# Autodesk Inventor assembly: StepperSystem
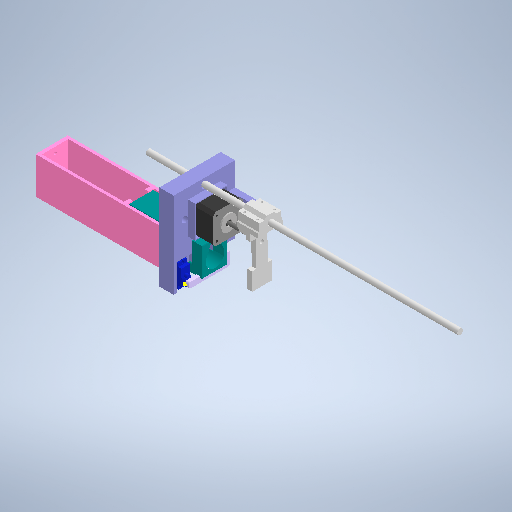
[picture p0: Inventor's stored thumbnail of the model, 512x512]
Saved by Autodesk Inventor 2025.1 (Build 291241000, 241)
## iProperties
Created: 2025-01-26
Part Number: StepperSystem
Document SubType Name: Assembly
Designer: 13156
Author: 13156
## Documents named in this file (10)
- C:\Users\13156\OneDrive - Binghamton University\Documents\GitHub\Perovskite-Automated-Synthesis-System\CAD\Pipette\StepperSystem.iam
- C:\Users\13156\OneDrive - Binghamton University\Documents\GitHub\Perovskite-Automated-Synthesis-System\CAD\Pipette\HolderWStepper.ipt
- C:\Users\13156\OneDrive - Binghamton University\Documents\GitHub\Perovskite-Automated-Synthesis-System\CAD\Non 3D Printed Parts\Motors and Servos\NEMA17 Stepper Motor.ipt
- C:\Users\13156\OneDrive - Binghamton University\Documents\GitHub\Perovskite-Automated-Synthesis-System\CAD\Non 3D Printed Parts\Linear Rails\8mm Linear Rod.ipt
- C:\Users\13156\OneDrive - Binghamton University\Documents\GitHub\Perovskite-Automated-Synthesis-System\CAD\Non 3D Printed Parts\Linear Rails\Linear Bearing 8mm Square.ipt
- C:\Users\13156\OneDrive - Binghamton University\Documents\GitHub\Perovskite-Automated-Synthesis-System\CAD\Pipette\Actuator.ipt
- C:\Users\13156\OneDrive - Binghamton University\Documents\GitHub\Perovskite-Automated-Synthesis-System\CAD\Pipette\PipetteSleeveFullLength.ipt
- C:\Users\13156\OneDrive - Binghamton University\Documents\GitHub\Perovskite-Automated-Synthesis-System\CAD\Pipette\PipetteStand.ipt
- C:\Users\13156\OneDrive - Binghamton University\Documents\GitHub\Perovskite-Automated-Synthesis-System\CAD\Non 3D Printed Parts\Motors and Servos\SG90 Servo.ipt
- C:\Users\13156\OneDrive - Binghamton University\Documents\GitHub\Perovskite-Automated-Synthesis-System\CAD\Pipette\GrabberArm.ipt
## Components (9 placed, 9 different names)
1. HolderWStepper:1 — Mate:1, Angle:1, Mate:4
2. NEMA17 Stepper Motor:1 — Mate:1
3. 8mm Linear Rod:1 — Angle:1, Mate:2
4. Linear Bearing 8mm Square:1 — Mate:2
5. Actuator:1
6. PipetteSleeveFullLength:1 — Mate:3
7. PipetteStand:1 — Mate:3
8. SG90 Servo:1 — Mate:4, Mate:5, Mate:6
9. GrabberArm:1 — Mate:5, Mate:6
## Relationships (7: Mate 6, Angle 1)
- Mate:1: HolderWStepper:1 ↔ NEMA17 Stepper Motor:1
- Angle:1 (0 deg): HolderWStepper:1 ↔ 8mm Linear Rod:1
- Mate:2: 8mm Linear Rod:1 ↔ Linear Bearing 8mm Square:1
- Mate:3: PipetteSleeveFullLength:1 ↔ PipetteStand:1
- Mate:4: HolderWStepper:1 ↔ SG90 Servo:1
- Mate:5: SG90 Servo:1 ↔ GrabberArm:1
- Mate:6: SG90 Servo:1 ↔ GrabberArm:1
